# Autodesk Inventor assembly: LuEvo5
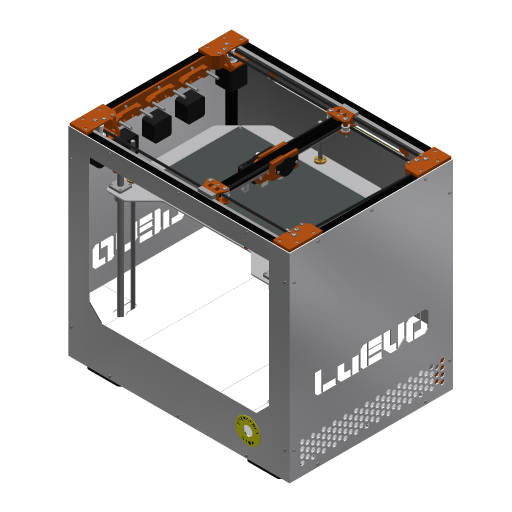
[picture p0: Inventor's stored thumbnail of the model, 512x512]
Saved by Autodesk Inventor 2023.2 (Build 272271000, 271)
## iProperties
Created: 2023-02-02
Part Number: LuEvo5
Document SubType Name: Assembly
Designer: remop
Author: remop
## Documents named in this file (26)
- C:\Users\remop\OneDrive\Documents\Inventor\3D Printers\LuEVO\Mk5_FullKinematic\LuEvo5.iam
- C:\Users\remop\OneDrive\Documents\Inventor\3D Printers\LuEVO\Mk5_FullKinematic\Mk5_BottomFrame.iam
- C:\Users\remop\OneDrive\Documents\Inventor\3D Printers\LuEVO\Mk5_FullKinematic\Mk5_TopFrame.iam
- C:\Users\remop\OneDrive\Documents\Inventor\3D Printers\LuEVO\Mk5_FullKinematic\Z Axis Front Right.iam
- C:\Users\remop\OneDrive\Documents\Inventor\3D Printers\LuEVO\Mk5_FullKinematic\Z Axis Front Left.iam
- C:\Users\remop\OneDrive\Documents\Inventor\3D Printers\LuEVO\Mk5_FullKinematic\Z Axis Rear.iam
- C:\Users\remop\OneDrive\Documents\Inventor\3D Printers\LuEVO\Mk5_FullKinematic\Z Axis.iam
- C:\Users\remop\OneDrive\Documents\Inventor\3D Printers\LuEVO\Mk5_FullKinematic\MGNR12_500mm.ipt
- C:\Users\remop\OneDrive\Documents\Inventor\3D Printers\LuEVO\Mk5_FullKinematic\Y Axis.iam
- C:\Users\remop\OneDrive\Documents\Inventor\3D Printers\LuEVO\Mk5_FullKinematic\Extruder Carriage.iam
- C:\Users\remop\OneDrive\Documents\Inventor\Content Center Files\R2023\en-US\AS 1420\AS 1420 - 1973 - M3 x 8.ipt
- C:\Users\remop\OneDrive\Documents\Inventor\3D Printers\LuEVO\Mk5_FullKinematic\Alpha Motor Assembly.iam
- C:\Users\remop\OneDrive\Documents\Inventor\3D Printers\LuEVO\Mk5_FullKinematic\Beta Motor Assembly.iam
- C:\Users\remop\OneDrive\Documents\Inventor\3D Printers\LuEVO\Mk5_FullKinematic\Alpha Idler Assembly.iam
- C:\Users\remop\OneDrive\Documents\Inventor\3D Printers\LuEVO\Mk5_FullKinematic\Beta Idler Assembly.iam
- C:\Users\remop\OneDrive\Documents\Inventor\3D Printers\LuEVO\Mk3\TopBrace.ipt
- C:\Users\remop\OneDrive\Documents\Inventor\3D Printers\LuEVO\Mk5_FullKinematic\Belt_1.ipt
- C:\Users\remop\OneDrive\Documents\Inventor\3D Printers\LuEVO\Mk5_FullKinematic\Belt_2.ipt
- C:\Users\remop\OneDrive\Documents\Inventor\3D Printers\LuEVO\Mk5_FullKinematic\Lightbar Assembly.iam
- C:\Users\remop\OneDrive\Documents\Inventor\3D Printers\LuEVO\Mk5_FullKinematic\Extruder Side Panel Assembly.iam
- C:\Users\remop\OneDrive\Documents\Inventor\3D Printers\LuEVO\Mk5_FullKinematic\Tool Dock Assembly.iam
- C:\Users\remop\OneDrive\Documents\Inventor\3D Printers\LuEVO\Mk4_Toolchanger\MagToolChanger_Tool.iam
- C:\Users\remop\OneDrive\Documents\Inventor\3D Printers\LuEVO\Mk5_FullKinematic\Camera Side Panel Assembly.iam
- C:\Users\remop\OneDrive\Documents\Inventor\3D Printers\LuEVO\Mk5_FullKinematic\Rear Panel Assembly.iam
- C:\Users\remop\OneDrive\Documents\Inventor\3D Printers\LuEVO\Mk5_FullKinematic\Front Panel Assembly.iam
- C:\Users\remop\OneDrive\Documents\Inventor\3D Printers\LuEVO\Mk5_FullKinematic\Electronics Cover.ipt
## Components (71 placed, 25 different names)
1. Bottom Frame [sub-assembly] — Rotational:1, Rotational:2, Mate:4
2. Top Frame [sub-assembly] — Rotational:1, Rotational:2, Flush:1, Mate:1, Flush:2, Flush:3, Flush:4, Mate:2, Mate:3, Flush:5, Mate:5, Flush:6, Mate:6, Mate:7, Mate:8, Flush:7, Mate:14, Flush:8, Flush:9, Mate:15, Flush:11, Flush:12, Flush:13, Flush:14, Mate:16, Flush:15, Flush:16, Mate:17, Flush:17, Flush:18, Flush:19, Mate:18, Mate:23, Mate:29, Flush:22, Mate:30, Flush:23, Flush:25, Flush:26, Mate:32, Mate:33, Mate:34, Mate:37, Mate:38, Mate:39, Flush:29
3. Z Axis Front Right [sub-assembly] — Flush:1, Mate:1, Flush:2, Mate:31
4. Z Axis Front Left [sub-assembly] — Flush:3, Flush:4, Mate:2
5. Z Axis Rear [sub-assembly] — Mate:3, Flush:5, Mate:4
6. Z Axis [sub-assembly]
7. MGNR12_500mm:1 — Mate:5, Flush:6, Mate:6, Insert:9, Insert:10, Insert:11, Insert:12, Insert:13, Insert:14, Insert:15, Insert:16, Insert:17, Insert:18, Insert:19, Insert:20, Insert:21, Insert:22, Insert:23, Insert:24, Insert:25, Insert:26, Insert:27, Insert:28
8. MGNR12_500mm:2 — Mate:7, Mate:8, Flush:7, Mate:9, Mate:10, Insert:29, Insert:30, Insert:31, Insert:32, Insert:33, Insert:34, Insert:35, Insert:36, Insert:37, Insert:38, Insert:39, Insert:40, Insert:41, Insert:42, Insert:43, Insert:44, Insert:45, Insert:46, Insert:47, Insert:48
9. Gantry [sub-assembly] — Mate:9, Mate:10, Mate:12, Mate:13, Insert:1, Insert:2, Insert:3, Insert:4, Mate:23, Mate:24, Mate:25, Mate:26, Mate:27
10. Extruder Carriage:1 [sub-assembly] — Mate:12, Mate:13, Mate:24, Flush:27, Flush:28, Mate:36
11. Alpha Motor Assembly [sub-assembly] — Mate:14, Flush:8, Flush:9, Mate:28
12. Beta Motor Assembly [sub-assembly] — Mate:15, Flush:11, Flush:12, Mate:35
13. Alpha Idler Assembly:1 [sub-assembly] — Flush:13, Flush:14, Mate:16
14. Beta Idler Assembly:1 [sub-assembly] — Flush:15, Flush:16, Mate:17
15. TopBrace:1 — Flush:17, Flush:18, Flush:20, Flush:21
16. TopBrace:2 — Flush:19, Flush:20, Flush:21, Mate:18
17. Belt_1:1 — Mate:25
18. Belt_2:1 — Mate:26, Mate:27, Mate:28
19. Lightbar Assembly:1 [sub-assembly] — Mate:29, Flush:22, Flush:24
20. Lightbar Assembly:2 [sub-assembly] — Mate:30, Flush:23, Mate:31, Flush:24
21. Tool Dock Assembly:1 [sub-assembly] — Mate:33, Mate:34, Mate:35
22. MagToolChanger_Tool:1 [sub-assembly] — Flush:27, Flush:28, Mate:36
23. Extruder Side Panel Assembly:1 [sub-assembly] — Flush:25, Flush:26, Mate:32
24. Camera Side Panel Assembly:1 [sub-assembly] — Mate:37
25. Rear Panel Assembly:1 [sub-assembly] — Mate:38
26. Front Panel Assembly:1 [sub-assembly] — Mate:39
27. Electronics Cover:1 — Flush:29
28. AS 1420 - Metric M3 x 8:1 — Insert:1
29. AS 1420 - Metric M3 x 8:2 — Insert:2
30. AS 1420 - Metric M3 x 8:3 — Insert:3
31. AS 1420 - Metric M3 x 8:4 — Insert:4
32. AS 1420 - Metric M3 x 8:5 — Insert:9
33. AS 1420 - Metric M3 x 8:6 — Insert:10
34. AS 1420 - Metric M3 x 8:7 — Insert:11
35. AS 1420 - Metric M3 x 8:8 — Insert:12
36. AS 1420 - Metric M3 x 8:9 — Insert:13
37. AS 1420 - Metric M3 x 8:10 — Insert:14
38. AS 1420 - Metric M3 x 8:11 — Insert:15
39. AS 1420 - Metric M3 x 8:12 — Insert:16
40. AS 1420 - Metric M3 x 8:13 — Insert:17
41. AS 1420 - Metric M3 x 8:14 — Insert:18
42. AS 1420 - Metric M3 x 8:15 — Insert:19
43. AS 1420 - Metric M3 x 8:16 — Insert:20
44. AS 1420 - Metric M3 x 8:17 — Insert:21
45. AS 1420 - Metric M3 x 8:18 — Insert:22
46. AS 1420 - Metric M3 x 8:19 — Insert:23
47. AS 1420 - Metric M3 x 8:20 — Insert:24
48. AS 1420 - Metric M3 x 8:21 — Insert:25
49. AS 1420 - Metric M3 x 8:22 — Insert:26
50. AS 1420 - Metric M3 x 8:23 — Insert:27
51. AS 1420 - Metric M3 x 8:24 — Insert:28
52. AS 1420 - Metric M3 x 8:25 — Insert:29
53. AS 1420 - Metric M3 x 8:26 — Insert:30
54. AS 1420 - Metric M3 x 8:27 — Insert:31
55. AS 1420 - Metric M3 x 8:28 — Insert:32
56. AS 1420 - Metric M3 x 8:29 — Insert:33
57. AS 1420 - Metric M3 x 8:30 — Insert:34
58. AS 1420 - Metric M3 x 8:31 — Insert:35
59. AS 1420 - Metric M3 x 8:32 — Insert:36
60. AS 1420 - Metric M3 x 8:33 — Insert:37
61. AS 1420 - Metric M3 x 8:34 — Insert:38
62. AS 1420 - Metric M3 x 8:35 — Insert:39
63. AS 1420 - Metric M3 x 8:36 — Insert:40
64. AS 1420 - Metric M3 x 8:37 — Insert:41
65. AS 1420 - Metric M3 x 8:38 — Insert:42
66. AS 1420 - Metric M3 x 8:39 — Insert:43
67. AS 1420 - Metric M3 x 8:40 — Insert:44
68. AS 1420 - Metric M3 x 8:41 — Insert:45
69. AS 1420 - Metric M3 x 8:42 — Insert:46
70. AS 1420 - Metric M3 x 8:43 — Insert:47
71. AS 1420 - Metric M3 x 8:44 — Insert:48
## Relationships (108: Insert 44, Mate 34, Flush 28, RevoluteJoint 2)
- Rotational:1 [RevoluteJoint]: Bottom Frame ↔ Top Frame
- Rotational:2 [RevoluteJoint]: Bottom Frame ↔ Top Frame
- Flush:1: Top Frame ↔ Z Axis Front Right
- Mate:1: Top Frame ↔ Z Axis Front Right
- Flush:2: Top Frame ↔ Z Axis Front Right
- Flush:3: Top Frame ↔ Z Axis Front Left
- Flush:4: Top Frame ↔ Z Axis Front Left
- Mate:2: Top Frame ↔ Z Axis Front Left
- Mate:3: Top Frame ↔ Z Axis Rear
- Flush:5: Top Frame ↔ Z Axis Rear
- Mate:4 (80.5 mm): Bottom Frame ↔ Z Axis Rear
- Mate:5: Top Frame ↔ MGNR12_500mm:1
- Flush:6 (1.5 mm): Top Frame ↔ MGNR12_500mm:1
- Mate:6: Top Frame ↔ MGNR12_500mm:1
- Mate:7: Top Frame ↔ MGNR12_500mm:2
- Mate:8: Top Frame ↔ MGNR12_500mm:2
- Flush:7 (1.5 mm): Top Frame ↔ MGNR12_500mm:2
- Mate:9: MGNR12_500mm:2 ↔ Gantry
- Mate:10: MGNR12_500mm:2 ↔ Gantry
- Mate:12: Gantry ↔ Extruder Carriage:1
- Mate:13: Gantry ↔ Extruder Carriage:1
- Insert:1: Gantry ↔ AS 1420 - Metric M3 x 8:1
- Insert:2: Gantry ↔ AS 1420 - Metric M3 x 8:2
- Insert:3: Gantry ↔ AS 1420 - Metric M3 x 8:3
- Insert:4: Gantry ↔ AS 1420 - Metric M3 x 8:4
- Insert:9: MGNR12_500mm:1 ↔ AS 1420 - Metric M3 x 8:5
- Insert:10: MGNR12_500mm:1 ↔ AS 1420 - Metric M3 x 8:6
- Insert:11: MGNR12_500mm:1 ↔ AS 1420 - Metric M3 x 8:7
- Insert:12: MGNR12_500mm:1 ↔ AS 1420 - Metric M3 x 8:8
- Insert:13: MGNR12_500mm:1 ↔ AS 1420 - Metric M3 x 8:9
- Insert:14: MGNR12_500mm:1 ↔ AS 1420 - Metric M3 x 8:10
- Insert:15: MGNR12_500mm:1 ↔ AS 1420 - Metric M3 x 8:11
- Insert:16: MGNR12_500mm:1 ↔ AS 1420 - Metric M3 x 8:12
- Insert:17: MGNR12_500mm:1 ↔ AS 1420 - Metric M3 x 8:13
- Insert:18: MGNR12_500mm:1 ↔ AS 1420 - Metric M3 x 8:14
- Insert:19: MGNR12_500mm:1 ↔ AS 1420 - Metric M3 x 8:15
- Insert:20: MGNR12_500mm:1 ↔ AS 1420 - Metric M3 x 8:16
- Insert:21: MGNR12_500mm:1 ↔ AS 1420 - Metric M3 x 8:17
- Insert:22: MGNR12_500mm:1 ↔ AS 1420 - Metric M3 x 8:18
- Insert:23: MGNR12_500mm:1 ↔ AS 1420 - Metric M3 x 8:19
- Insert:24: MGNR12_500mm:1 ↔ AS 1420 - Metric M3 x 8:20
- Insert:25: MGNR12_500mm:1 ↔ AS 1420 - Metric M3 x 8:21
- Insert:26: MGNR12_500mm:1 ↔ AS 1420 - Metric M3 x 8:22
- Insert:27: MGNR12_500mm:1 ↔ AS 1420 - Metric M3 x 8:23
- Insert:28: MGNR12_500mm:1 ↔ AS 1420 - Metric M3 x 8:24
- Insert:29: MGNR12_500mm:2 ↔ AS 1420 - Metric M3 x 8:25
- Insert:30: MGNR12_500mm:2 ↔ AS 1420 - Metric M3 x 8:26
- Insert:31: MGNR12_500mm:2 ↔ AS 1420 - Metric M3 x 8:27
- Insert:32: MGNR12_500mm:2 ↔ AS 1420 - Metric M3 x 8:28
- Insert:33: MGNR12_500mm:2 ↔ AS 1420 - Metric M3 x 8:29
- Insert:34: MGNR12_500mm:2 ↔ AS 1420 - Metric M3 x 8:30
- Insert:35: MGNR12_500mm:2 ↔ AS 1420 - Metric M3 x 8:31
- Insert:36: MGNR12_500mm:2 ↔ AS 1420 - Metric M3 x 8:32
- Insert:37: MGNR12_500mm:2 ↔ AS 1420 - Metric M3 x 8:33
- Insert:38: MGNR12_500mm:2 ↔ AS 1420 - Metric M3 x 8:34
- Insert:39: MGNR12_500mm:2 ↔ AS 1420 - Metric M3 x 8:35
- Insert:40: MGNR12_500mm:2 ↔ AS 1420 - Metric M3 x 8:36
- Insert:41: MGNR12_500mm:2 ↔ AS 1420 - Metric M3 x 8:37
- Insert:42: MGNR12_500mm:2 ↔ AS 1420 - Metric M3 x 8:38
- Insert:43: MGNR12_500mm:2 ↔ AS 1420 - Metric M3 x 8:39
- Insert:44: MGNR12_500mm:2 ↔ AS 1420 - Metric M3 x 8:40
- Insert:45: MGNR12_500mm:2 ↔ AS 1420 - Metric M3 x 8:41
- Insert:46: MGNR12_500mm:2 ↔ AS 1420 - Metric M3 x 8:42
- Insert:47: MGNR12_500mm:2 ↔ AS 1420 - Metric M3 x 8:43
- Insert:48: MGNR12_500mm:2 ↔ AS 1420 - Metric M3 x 8:44
- Mate:14: Top Frame ↔ Alpha Motor Assembly
- Flush:8: Top Frame ↔ Alpha Motor Assembly
- Flush:9: Top Frame ↔ Alpha Motor Assembly
- Mate:15: Top Frame ↔ Beta Motor Assembly
- Flush:11: Top Frame ↔ Beta Motor Assembly
- Flush:12: Top Frame ↔ Beta Motor Assembly
- Flush:13: Top Frame ↔ Alpha Idler Assembly:1
- Flush:14: Top Frame ↔ Alpha Idler Assembly:1
- Mate:16: Top Frame ↔ Alpha Idler Assembly:1
- Flush:15: Top Frame ↔ Beta Idler Assembly:1
- Flush:16: Top Frame ↔ Beta Idler Assembly:1
- Mate:17: Top Frame ↔ Beta Idler Assembly:1
- Flush:17: Top Frame ↔ TopBrace:1
- Flush:18: Top Frame ↔ TopBrace:1
- Flush:19: Top Frame ↔ TopBrace:2
- Flush:20: TopBrace:1 ↔ TopBrace:2
- Flush:21: TopBrace:1 ↔ TopBrace:2
- Mate:18 (10 mm): Top Frame ↔ TopBrace:2
- Mate:23 (200 mm): Top Frame ↔ Gantry
- Mate:24 (106.7 mm): Gantry ↔ Extruder Carriage:1
- Mate:25 (0.5 mm): Gantry ↔ Belt_1:1
- Mate:26 (0.5 mm): Gantry ↔ Belt_2:1
- Mate:27: Gantry ↔ Belt_2:1
- Mate:28: Alpha Motor Assembly ↔ Belt_2:1
- Mate:29: Top Frame ↔ Lightbar Assembly:1
- Flush:22: Top Frame ↔ Lightbar Assembly:1
- Mate:30: Top Frame ↔ Lightbar Assembly:2
- Flush:23: Top Frame ↔ Lightbar Assembly:2
- Mate:31 (5.5 mm): Z Axis Front Right ↔ Lightbar Assembly:2
- Flush:24: Lightbar Assembly:1 ↔ Lightbar Assembly:2
- Flush:25: Top Frame ↔ Extruder Side Panel Assembly:1
- Flush:26: Top Frame ↔ Extruder Side Panel Assembly:1
- Mate:32: Top Frame ↔ Extruder Side Panel Assembly:1
- Mate:33: Top Frame ↔ Tool Dock Assembly:1
- Mate:34: Top Frame ↔ Tool Dock Assembly:1
- Mate:35 (2.5 mm): Beta Motor Assembly ↔ Tool Dock Assembly:1
- Flush:27: Extruder Carriage:1 ↔ MagToolChanger_Tool:1
- Flush:28: Extruder Carriage:1 ↔ MagToolChanger_Tool:1
- Mate:36 (1 mm): Extruder Carriage:1 ↔ MagToolChanger_Tool:1
- Mate:37: Top Frame ↔ Camera Side Panel Assembly:1
- Mate:38: Top Frame ↔ Rear Panel Assembly:1
- Mate:39: Top Frame ↔ Front Panel Assembly:1
- Flush:29: Top Frame ↔ Electronics Cover:1
